# Autodesk Inventor assembly: ASY PNS-0100 MAIN FRAME
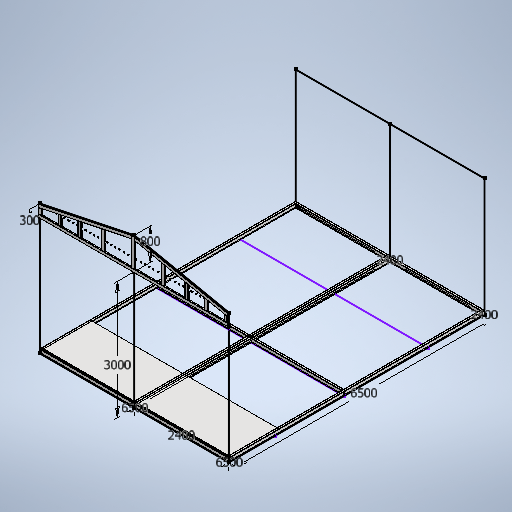
[picture p0: Inventor's stored thumbnail of the model, 512x512]
Saved by Autodesk Inventor 2025 (Build 290162010, 162A)
## iProperties
Created: 2025-03-10
Part Number: ASY PNS-0100 MAIN FRAME
Document SubType Name: Assembly
Designer: admin
Author: admin
## Documents named in this file (4)
- C:\Users\admin\YandexDisk-badmisterfox\home pc\Inventor\PNS-Panaevsk\ASY PNS-0100 MAIN FRAME.iam
- C:\Users\admin\YandexDisk-badmisterfox\home pc\Inventor\PNS-Panaevsk\PNS-0100 FRAME Main sketch.ipt
- C:\Users\admin\YandexDisk-badmisterfox\home pc\Inventor\PNS-Panaevsk\ASY PNS-0110 frame left floor.iam
- C:\Users\admin\YandexDisk-badmisterfox\home pc\Inventor\PNS-Panaevsk\ASY PNS-0170 frame roof.iam
## Components (4 placed, 3 different names)
1. PNS-0100 FRAME Main sketch:1
2. ASY PNS-0110 frame left floor:1 [sub-assembly] — Flush:1, Flush:2, Flush:3, Rigid:1
3. ASY PNS-0110 frame left floor:2 [sub-assembly] — Rigid:1
4. ASY PNS-0170 frame roof:1 [sub-assembly]
## Relationships (4: Flush 3, WeldJoint 1)
- Flush:1: ASY PNS-0110 frame left floor:1
- Flush:2: ASY PNS-0110 frame left floor:1
- Flush:3: ASY PNS-0110 frame left floor:1
- Rigid:1 [WeldJoint]: ASY PNS-0110 frame left floor:1 ↔ ASY PNS-0110 frame left floor:2
